# Autodesk Inventor assembly: Wing Right
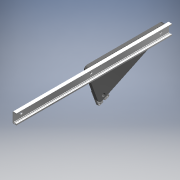
[picture p0: Inventor's stored thumbnail of the model, 180x180]
Saved by Autodesk Inventor 2019 (Build 230136000, 136)
## iProperties
Part Number: Wing Right
Document SubType Name: Assembly
Designer: Delta
Author: Delta
## Documents named in this file (4)
- C:\Robotics\2019-20_CAD\Collection\Wing Right.iam
- C:\Robotics\COTSParts\Misumi_Slides\AIS2018\SAR330-30_b.ipt
- C:\Robotics\2019-20_CAD\Collection\Triangle axle slide connector.ipt
- C:\Robotics\COTSParts\Rev\REV-41-1683 Bear Blocks.ipt
## Components (3 placed, 3 different names)
1. SAR330-30_b:1 — Flush:1, Mate:1, Mate:2
2. Triangle axle slide connector:1 — Flush:1, Mate:1, Mate:2, Mate:3, Angle:1
3. REV-41-1683 Bear Blocks:1 — Mate:3, Angle:1
## Relationships (5: Mate 3, Flush 1, Angle 1)
- Flush:1: SAR330-30_b:1 ↔ Triangle axle slide connector:1
- Mate:1: SAR330-30_b:1 ↔ Triangle axle slide connector:1
- Mate:2 (0.01 mm): SAR330-30_b:1 ↔ Triangle axle slide connector:1
- Mate:3: Triangle axle slide connector:1 ↔ REV-41-1683 Bear Blocks:1
- Angle:1 (0 deg): Triangle axle slide connector:1 ↔ REV-41-1683 Bear Blocks:1
